# Autodesk Inventor assembly: trzymak
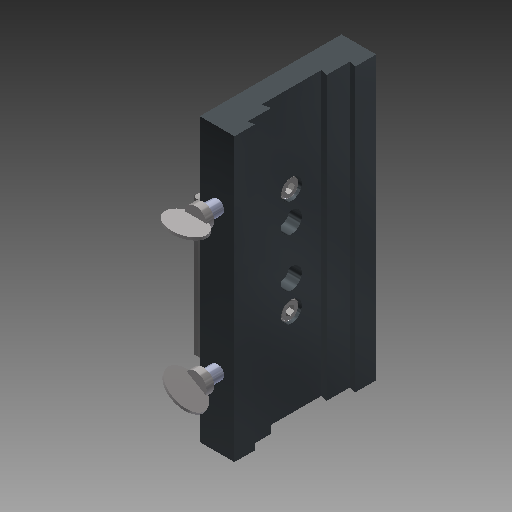
[picture p0: Inventor's stored thumbnail of the model, 512x512]
Saved by Autodesk Inventor 2019.4 (Build 234330000, 330)
## iProperties
Created: 2020-08-30
Part Number: trzymak
Document SubType Name: Assembly
Designer: estee
Author: estee
## Documents named in this file (7)
- F:\GitHub\MUMv2\Equatorial-Mount-MUM\Mechanika\Moduł obrotu RET Estera\prawieKoncowka\trzymak.iam
- F:\GitHub\MUMv2\Equatorial-Mount-MUM\Mechanika\Moduł obrotu RET Estera\prawieKoncowka\plytkaadaptacyjna.ipt
- F:\GitHub\MUMv2\Equatorial-Mount-MUM\Mechanika\Moduł obrotu RET Estera\prawieKoncowka\uchwytDoSzyny.iam
- F:\GitHub\MUMv2\Equatorial-Mount-MUM\Mechanika\Moduł obrotu RET Estera\prawieKoncowka\kolnierz.ipt
- F:\GitHub\MUMv2\Equatorial-Mount-MUM\Mechanika\Moduł obrotu RET Estera\prawieKoncowka\ISO 4762 - M8 x 20ISO.ipt
- F:\GitHub\MUMv2\Equatorial-Mount-MUM\Mechanika\Moduł obrotu RET Estera\prawieKoncowka\ISO 4032 - M8 - ISO.ipt
- F:\GitHub\MUMv2\Equatorial-Mount-MUM\Mechanika\Moduł obrotu RET Estera\prawieKoncowka\ISO 7046-1 - M3 x 8 - 4.8 - Z - ISO.ipt
## Components (11 placed, 6 different names)
1. plytkaadaptacyjna:1 — Mate:1, Mate:2, Mate:3, Mate:12, Mate:13, Mate:14, Mate:19, Mate:20, Mate:23, Mate:24, Mate:25, Mate:26, Flush:1, Flush:2, Flush:3, Flush:4
2. uchwytDoSzyny:1 [sub-assembly] — Mate:12, Mate:13, Mate:14, Mate:15, Mate:16, Mate:17, Mate:18, Mate:27, Flush:5
3. kolnierz:2 — Mate:1, Mate:2, Mate:3
4. ISO 4762 M8 x 20:1 — Mate:17, Mate:18, Mate:22
5. ISO 4762 M8 x 20:2 — Mate:15, Mate:16
6. ISO 4032 M8:1 — Mate:19, Mate:22
7. ISO 4032 M8:2 — Mate:20
8. ISO 7046-1 Z M3 x 8 - 4.8 - Z:2 — Mate:23, Flush:1
9. ISO 7046-1 Z M3 x 8 - 4.8 - Z:3 — Mate:25, Flush:4
10. ISO 7046-1 Z M3 x 8 - 4.8 - Z:4 — Mate:26, Flush:2
11. ISO 7046-1 Z M3 x 8 - 4.8 - Z:5 — Mate:24, Flush:3
## Relationships (23: Mate 18, Flush 5)
- Mate:1: plytkaadaptacyjna:1 ↔ kolnierz:2
- Mate:2: plytkaadaptacyjna:1 ↔ kolnierz:2
- Mate:3: plytkaadaptacyjna:1 ↔ kolnierz:2
- Mate:12: plytkaadaptacyjna:1 ↔ uchwytDoSzyny:1
- Mate:13: plytkaadaptacyjna:1 ↔ uchwytDoSzyny:1
- Mate:14: plytkaadaptacyjna:1 ↔ uchwytDoSzyny:1
- Mate:15: uchwytDoSzyny:1 ↔ ISO 4762 M8 x 20:2
- Mate:16: uchwytDoSzyny:1 ↔ ISO 4762 M8 x 20:2
- Mate:17: uchwytDoSzyny:1 ↔ ISO 4762 M8 x 20:1
- Mate:18: uchwytDoSzyny:1 ↔ ISO 4762 M8 x 20:1
- Mate:19: plytkaadaptacyjna:1 ↔ ISO 4032 M8:1
- Mate:20: plytkaadaptacyjna:1 ↔ ISO 4032 M8:2
- Mate:22: ISO 4762 M8 x 20:1 ↔ ISO 4032 M8:1
- Mate:23: plytkaadaptacyjna:1 ↔ ISO 7046-1 Z M3 x 8 - 4.8 - Z:2
- Mate:24: plytkaadaptacyjna:1 ↔ ISO 7046-1 Z M3 x 8 - 4.8 - Z:5
- Mate:25: plytkaadaptacyjna:1 ↔ ISO 7046-1 Z M3 x 8 - 4.8 - Z:3
- Mate:26: plytkaadaptacyjna:1 ↔ ISO 7046-1 Z M3 x 8 - 4.8 - Z:4
- Flush:1: plytkaadaptacyjna:1 ↔ ISO 7046-1 Z M3 x 8 - 4.8 - Z:2
- Flush:2: plytkaadaptacyjna:1 ↔ ISO 7046-1 Z M3 x 8 - 4.8 - Z:4
- Flush:3: plytkaadaptacyjna:1 ↔ ISO 7046-1 Z M3 x 8 - 4.8 - Z:5
- Flush:4: plytkaadaptacyjna:1 ↔ ISO 7046-1 Z M3 x 8 - 4.8 - Z:3
- Mate:27: uchwytDoSzyny:1
- Flush:5: uchwytDoSzyny:1
